# Autodesk Inventor assembly: ExteriorBumperCar2
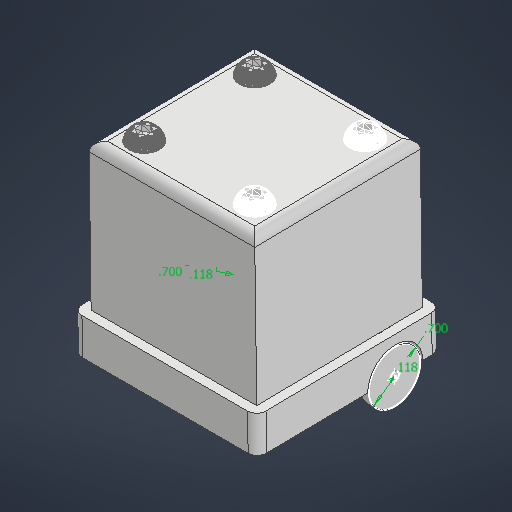
[picture p0: Inventor's stored thumbnail of the model, 512x512]
Saved by Autodesk Inventor 2026.1 (Build 301233000, 233)
## iProperties
Created: 2026-06-28
Part Number: ExteriorBumperCar2
Document SubType Name: Assembly
Designer: Kasi Pusuluri
Author: Kasi Pusuluri
## Documents named in this file (12)
- C:\Users\Kasi Pusuluri\Documents\Outpost 2026\BumperCarV2\ExteriorBumperCar2.iam
- C:\Users\Kasi Pusuluri\Documents\Outpost 2026\BumperCarV2\BumperBody.ipt
- C:\Users\Kasi Pusuluri\Documents\Outpost 2026\BumperCarV2\WheelAssembly.iam
- C:\Users\Kasi Pusuluri\Documents\Outpost 2026\BumperCarV2\BumperCaster2.ipt
- C:\Users\Kasi Pusuluri\Documents\Outpost 2026\BumperCarV2\Base.ipt
- C:\Users\Kasi Pusuluri\Documents\Outpost 2026\BumperCarV2\Battery2.ipt
- C:\Users\Kasi Pusuluri\Documents\Outpost 2026\BumperCarV2\WheelConnector.ipt
- C:\Users\Kasi Pusuluri\Documents\Outpost 2026\BumperCarV2\NRF24L01+.ipt
- C:\Users\Kasi Pusuluri\Documents\Outpost 2026\BumperCarV2\Batteryyyy.ipt
- C:\Users\Kasi Pusuluri\Documents\Outpost 2026\BumperCarV2\Top.ipt
- C:\Users\Kasi Pusuluri\Documents\Outpost 2026\BumperCarV2\TopScrew.ipt
- C:\Users\Kasi Pusuluri\Documents\Outpost 2026\BumperCarV2\Connector1.ipt
## Components (19 placed, 11 different names)
1. BumperBody:1 — Mate:3, Mate:4, Mate:5, Mate:6, Mate:9, Mate:10, Mate:11
2. WheelAssembly:1 [sub-assembly] — Mate:4, Mate:6
3. WheelAssembly:2 [sub-assembly] — Mate:3, Mate:5, Mate:7, Mate:8
4. BumperCaster2:1 — Rotational:9
5. Base:1 — Mate:7, Mate:8, Rotational:9
6. Battery2:1
7. WheelConnector:1
8. WheelConnector:2
9. NRF24L01+:1
10. Batteryyyy:1
11. Top:1 — Rotational:10, Rotational:11, Rotational:12, Rotational:13, Rotational:14, Rotational:15, Rotational:16, Rotational:17, Mate:9, Mate:10, Mate:11
12. TopScrew:1 — Rotational:14
13. TopScrew:2 — Rotational:17
14. TopScrew:3 — Rotational:15
15. TopScrew:4 — Rotational:16
16. Connector1:1 — Rotational:10
17. Connector1:2 — Rotational:11
18. Connector1:3 — Rotational:12
19. Connector1:4 — Rotational:13
## Relationships (18: Mate 9, RevoluteJoint 9)
- Mate:3: BumperBody:1 ↔ WheelAssembly:2
- Mate:4: BumperBody:1 ↔ WheelAssembly:1
- Mate:5: BumperBody:1 ↔ WheelAssembly:2
- Mate:6: BumperBody:1 ↔ WheelAssembly:1
- Mate:7: WheelAssembly:2 ↔ Base:1
- Mate:8: WheelAssembly:2 ↔ Base:1
- Rotational:9 [RevoluteJoint]: BumperCaster2:1 ↔ Base:1
- Rotational:10 [RevoluteJoint]: Top:1 ↔ Connector1:1
- Rotational:11 [RevoluteJoint]: Top:1 ↔ Connector1:2
- Rotational:12 [RevoluteJoint]: Top:1 ↔ Connector1:3
- Rotational:13 [RevoluteJoint]: Top:1 ↔ Connector1:4
- Rotational:14 [RevoluteJoint]: Top:1 ↔ TopScrew:1
- Rotational:15 [RevoluteJoint]: Top:1 ↔ TopScrew:3
- Rotational:16 [RevoluteJoint]: Top:1 ↔ TopScrew:4
- Rotational:17 [RevoluteJoint]: Top:1 ↔ TopScrew:2
- Mate:9: BumperBody:1 ↔ Top:1
- Mate:10: BumperBody:1 ↔ Top:1
- Mate:11: BumperBody:1 ↔ Top:1
